# Autodesk Inventor assembly: will asembly
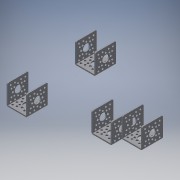
[picture p0: Inventor's stored thumbnail of the model, 180x180]
Saved by Autodesk Inventor 2019 (Build 230136000, 136)
## iProperties
Created: 2018-12-18
Part Number: will asembly
Document SubType Name: Assembly
Designer: User
Author: User
## Documents named in this file (2)
- C:\Robotics\CAD\2018-19_CAD\will\will asembly.iam
- C:\Robotics\CAD\COTSParts\Actobotics\585 parts\585440Channel1.5in.ipt
## Components (4 placed, 1 different names)
1. 585440Channel1.5in:1 — Mate:1
2. 585440Channel1.5in:2 — Mate:1
3. 585440Channel1.5in:3
4. 585440Channel1.5in:4
## Relationships (1: Mate 1)
- Mate:1: 585440Channel1.5in:1 ↔ 585440Channel1.5in:2
